# Autodesk Inventor assembly: leg_1
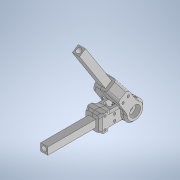
[picture p0: Inventor's stored thumbnail of the model, 180x180]
Saved by Autodesk Inventor 2020 (Build 240168000, 168)
## iProperties
Created: 2019-05-01
Part Number: leg_1
Document SubType Name: Assembly
Designer: psrob
Author: psrob
## Documents named in this file (5)
- E:\projects-2\project dog gen2\hardware\leg_1.iam
- E:\projects-2\project dog gen2\hardware\leg_bone_2.ipt
- E:\projects-2\project dog gen2\hardware\carbon_fiber_6.ipt
- E:\projects-2\project dog gen2\hardware\leg_bone_3.ipt
- E:\projects-2\project dog gen2\hardware\bone_upper_1.ipt
## Components (6 placed, 4 different names)
1. carbon_fiber_6:1 — Mate:1, Mate:2, Mate:3
2. leg_bone_2:1 — Mate:1, Mate:2, Mate:3, Insert:1, Insert:2
3. leg_bone_3:1 — Insert:1, Insert:2, Flush:1, Insert:3
4. bone_upper_1:1 — Flush:1, Mate:4, Mate:5, Insert:3, Mate:6, Insert:4, Insert:5
5. carbon_fiber_6:2 — Mate:4, Mate:5, Mate:6
6. bone_upper_1:2 — Insert:4, Insert:5
## Relationships (12: Mate 6, Insert 5, Flush 1)
- Mate:1: carbon_fiber_6:1 ↔ leg_bone_2:1
- Mate:2: carbon_fiber_6:1 ↔ leg_bone_2:1
- Mate:3: carbon_fiber_6:1 ↔ leg_bone_2:1
- Insert:1: leg_bone_2:1 ↔ leg_bone_3:1
- Insert:2: leg_bone_2:1 ↔ leg_bone_3:1
- Flush:1: leg_bone_3:1 ↔ bone_upper_1:1
- Mate:4: bone_upper_1:1 ↔ carbon_fiber_6:2
- Mate:5: bone_upper_1:1 ↔ carbon_fiber_6:2
- Insert:3: leg_bone_3:1 ↔ bone_upper_1:1
- Mate:6: bone_upper_1:1 ↔ carbon_fiber_6:2
- Insert:4: bone_upper_1:1 ↔ bone_upper_1:2
- Insert:5: bone_upper_1:1 ↔ bone_upper_1:2
